# Autodesk Inventor assembly: Filament Board
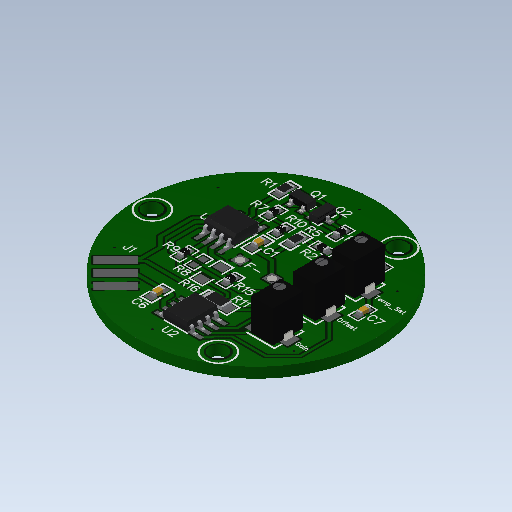
[picture p0: Inventor's stored thumbnail of the model, 512x512]
Saved by Autodesk Inventor 2020 (Build 240168000, 168)
## iProperties
Created: 2018-03-05
Part Number: Filament Board
Document SubType Name: Assembly
Designer: Alex
Description: Sensor Circuitry
Author: Alex
## Documents named in this file (10)
- C:\Users\amsmi\Google Drive\Pirani Gauge\Pirani Gauge Modeling\Gauge Rev 3\Filament Board.iam
- C:\Users\amsmi\Google Drive\Pirani Gauge\Pirani Gauge Modeling\Gauge Rev 3\Filament Board.ipt
- E:\Inventor Modeling\General Parts\Electronics\Surface Mount Components\SOIC8\sop127p-6mm-8 v2.iam
- E:\Inventor Modeling\General Parts\Electronics\Surface Mount Components\Black 0603.ipt
- E:\Inventor Modeling\General Parts\Electronics\Surface Mount Components\SOT23.iam
- E:\Inventor Modeling\General Parts\Electronics\Surface Mount Components\Cap 0603.ipt
- E:\Inventor Modeling\General Parts\Electronics\Surface Mount Components\Black 0805.ipt
- E:\Inventor Modeling\General Parts\Electronics\Surface Mount Components\Black 1206.ipt
- E:\Inventor Modeling\General Parts\Electronics\Surface Mount Components\SOT-23 (TO-236).ipt
- E:\Inventor Modeling\General Parts\Electronics\Surface Mount Components\SM42W.ipt
## Components (23 placed, 9 different names)
1. Filament Board:1 — Mate:1, Mate:2, Mate:3, Mate:10, Mate:11, Mate:14, Mate:15, Mate:17, Mate:18, Mate:19, Mate:21, Mate:22, Mate:23, Mate:24, Mate:25, Mate:26, Mate:27, Mate:28
2. sop127p-6mm-8 v2:1 [sub-assembly] — Flush:1, Mate:5, Mate:10, Mate:12, Mate:13, Flush:37
3. Black 0603:2 — Flush:8, Flush:9, Flush:30, Flush:31, Flush:34
4. Black 0603:3 — Flush:5, Flush:14, Flush:15, Flush:24, Flush:25, Flush:26, Flush:32, Flush:33, Flush:35
5. Black 0603:4 — Flush:4, Flush:5, Mate:11, Flush:14, Flush:15, Flush:34
6. Black 0603:5 — Flush:2, Mate:12, Mate:13, Flush:8, Flush:9, Flush:16, Flush:17, Flush:22, Flush:23, Angle:10
7. Black 0603:7 — Flush:2, Flush:4, Flush:16, Flush:17, Flush:28, Flush:29
8. SOT23:1 [sub-assembly] — Flush:18, Angle:7, Flush:19, Flush:20
9. SOT23:2 [sub-assembly] — Flush:18, Mate:14, Flush:21, Mate:16
10. Black 0603:8 — Mate:15, Flush:22, Flush:23, Flush:27
11. Cap 0603:1 — Mate:19, Angle:8, Angle:9, Flush:24, Flush:25
12. Cap 0603:2 — Mate:18, Angle:9, Flush:28, Flush:29
13. Black 0805:1 — Mate:17, Angle:10, Flush:26, Flush:27, Flush:35, Flush:36, Flush:38, Flush:39
14. Black 0805:2 — Mate:21, Flush:30, Flush:31, Flush:40, Flush:41
15. Black 1206:1 — Mate:22, Flush:32, Flush:33, Flush:48, Flush:49, Flush:52, Flush:53
16. Cap 0603:3 — Flush:36, Flush:37, Mate:23
17. Black 0603:9 — Mate:24, Flush:38, Flush:39
18. SOT-23 (TO-236):1 — Mate:26, Angle:11, Flush:42, Flush:43
19. SOT-23 (TO-236):2 — Mate:25, Flush:40, Flush:41, Angle:11, Flush:42, Flush:43
20. SM42W:1 — Flush:44, Flush:45, Flush:46, Flush:47, Flush:50, Flush:51
21. SM42W:2 — Flush:44, Mate:27, Flush:47, Flush:51
22. SM42W:3 — Flush:45, Flush:46, Flush:48, Flush:49, Flush:50, Angle:12
23. sop127p-6mm-8 v2:2 [sub-assembly] — Mate:28, Angle:12, Flush:52, Flush:53
## Relationships (74: Flush 46, Mate 22, Angle 6)
- Mate:1: Filament Board:1
- Mate:2: Filament Board:1
- Mate:3: Filament Board:1
- Flush:1 (7.1374 mm): sop127p-6mm-8 v2:1
- Mate:5 (-3.175 mm): sop127p-6mm-8 v2:1
- Mate:10: Filament Board:1 ↔ sop127p-6mm-8 v2:1
- Flush:2: Black 0603:5 ↔ Black 0603:7
- Flush:4: Black 0603:4 ↔ Black 0603:7
- Flush:5: Black 0603:3 ↔ Black 0603:4
- Mate:11: Filament Board:1 ↔ Black 0603:4
- Mate:12 (6.4262 mm): sop127p-6mm-8 v2:1 ↔ Black 0603:5
- Mate:13 (11.3538 mm): sop127p-6mm-8 v2:1 ↔ Black 0603:5
- Flush:8 (9.2456 mm): Black 0603:2 ↔ Black 0603:5
- Flush:9 (0.7366 mm): Black 0603:2 ↔ Black 0603:5
- Flush:14 (7.3406 mm): Black 0603:3 ↔ Black 0603:4
- Flush:15: Black 0603:3 ↔ Black 0603:4
- Flush:16 (6.6294 mm): Black 0603:5 ↔ Black 0603:7
- Flush:17 (2.3622 mm): Black 0603:5 ↔ Black 0603:7
- Flush:18: SOT23:1 ↔ SOT23:2
- Mate:14: Filament Board:1 ↔ SOT23:2
- Angle:7 (0 deg): SOT23:1
- Mate:15: Filament Board:1 ↔ Black 0603:8
- Flush:19 (12.3952 mm): SOT23:1
- Flush:20 (1.8034 mm): SOT23:1
- Flush:21 (5.2578 mm): SOT23:2
- Mate:16 (-12.7 mm): SOT23:2
- Flush:22 (3.2512 mm): Black 0603:5 ↔ Black 0603:8
- Flush:23 (-1.0922 mm): Black 0603:5 ↔ Black 0603:8
- Mate:17: Filament Board:1 ↔ Black 0805:1
- Mate:18: Filament Board:1 ↔ Cap 0603:2
- Mate:19: Filament Board:1 ↔ Cap 0603:1
- Angle:8 (90 deg): Cap 0603:1
- Angle:9 (0 deg): Cap 0603:1 ↔ Cap 0603:2
- Angle:10 (0 deg): Black 0603:5 ↔ Black 0805:1
- Flush:24 (-7.62 mm): Black 0603:3 ↔ Cap 0603:1
- Flush:25 (4.0132 mm): Black 0603:3 ↔ Cap 0603:1
- Flush:26 (-0.0254 mm): Black 0603:3 ↔ Black 0805:1
- Flush:27 (-4.7752 mm): Black 0603:8 ↔ Black 0805:1
- Flush:28 (-8.2042 mm): Black 0603:7 ↔ Cap 0603:2
- Flush:29 (4.953 mm): Black 0603:7 ↔ Cap 0603:2
- Mate:21: Filament Board:1 ↔ Black 0805:2
- Mate:22: Filament Board:1 ↔ Black 1206:1
- Flush:30 (3.81 mm): Black 0603:2 ↔ Black 0805:2
- Flush:31 (2.0828 mm): Black 0603:2 ↔ Black 0805:2
- Flush:32 (-4.064 mm): Black 0603:3 ↔ Black 1206:1
- Flush:33 (3.175 mm): Black 0603:3 ↔ Black 1206:1
- Flush:34 (1.4986 mm): Black 0603:2 ↔ Black 0603:4
- Flush:35 (-10.4902 mm): Black 0603:3 ↔ Black 0805:1
- Flush:36 (-3.2512 mm): Black 0805:1 ↔ Cap 0603:3
- Flush:37 (1.8288 mm): sop127p-6mm-8 v2:1 ↔ Cap 0603:3
- Mate:23: Filament Board:1 ↔ Cap 0603:3
- Mate:24: Filament Board:1 ↔ Black 0603:9
- Flush:38 (0.3302 mm): Black 0805:1 ↔ Black 0603:9
- Flush:39 (2.794 mm): Black 0805:1 ↔ Black 0603:9
- Mate:25: Filament Board:1 ↔ SOT-23 (TO-236):2
- Mate:26: Filament Board:1 ↔ SOT-23 (TO-236):1
- Flush:40 (0.2032 mm): Black 0805:2 ↔ SOT-23 (TO-236):2
- Flush:41 (4.1402 mm): Black 0805:2 ↔ SOT-23 (TO-236):2
- Angle:11 (90 deg): SOT-23 (TO-236):1 ↔ SOT-23 (TO-236):2
- Flush:42 (0.9906 mm): SOT-23 (TO-236):1 ↔ SOT-23 (TO-236):2
- Flush:43 (2.7432 mm): SOT-23 (TO-236):1 ↔ SOT-23 (TO-236):2
- Flush:44: SM42W:1 ↔ SM42W:2
- Flush:45: SM42W:1 ↔ SM42W:3
- Mate:27: Filament Board:1 ↔ SM42W:2
- Flush:46: SM42W:1 ↔ SM42W:3
- Flush:47: SM42W:1 ↔ SM42W:2
- Flush:48 (0.9652 mm): Black 1206:1 ↔ SM42W:3
- Flush:49 (-8.9916 mm): Black 1206:1 ↔ SM42W:3
- Flush:50 (-6.7564 mm): SM42W:1 ↔ SM42W:3
- Flush:51 (-6.2484 mm): SM42W:1 ↔ SM42W:2
- Mate:28: Filament Board:1 ↔ sop127p-6mm-8 v2:2
- Angle:12 (90 deg): SM42W:3 ↔ sop127p-6mm-8 v2:2
- Flush:52 (-5.715 mm): Black 1206:1 ↔ sop127p-6mm-8 v2:2
- Flush:53 (-1.4224 mm): Black 1206:1 ↔ sop127p-6mm-8 v2:2
